# Autodesk Inventor assembly: test rig
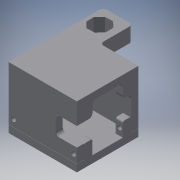
[picture p0: Inventor's stored thumbnail of the model, 180x180]
Saved by Autodesk Inventor 2016 (Build 200138000, 138)
## iProperties
Created: 2015-04-29
Part Number: test rig
Document SubType Name: Assembly
Designer: Jacob Kennedy
Author: Jacob Kennedy
## Documents named in this file (3)
- C:\Users\Jacob Kennedy\Documents\GitHub\Rocket Club Repo\RITLaunchInitiative\mechanical\TestEngine1\BallValveControl\Motor mount\test rig.iam
- C:\Users\Jacob Kennedy\Documents\new mount leftside.ipt
- C:\Users\Jacob Kennedy\Documents\new mount rightside.ipt
## Components (2 placed, 2 different names)
1. new mount leftside:1 — Flush:1
2. new mount rightside:1 — Flush:2
## Relationships (2: Flush 2)
- Flush:1: new mount leftside:1
- Flush:2: new mount rightside:1
